# Autodesk Inventor assembly: centre wing
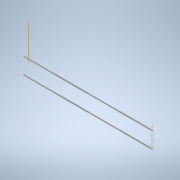
[picture p0: Inventor's stored thumbnail of the model, 180x180]
Saved by Autodesk Inventor 2022 (Build 260153000, 153)
## iProperties
Created: 2021-03-09
Part Number: centre wing
Document SubType Name: Assembly
Designer: Ferdinand Hubbard
Author: Ferdinand Hubbard
## Documents named in this file (4)
- C:\Users\Ferdinand Hubbard\Desktop\solar-plane\cad\centre wing section.iam
- C:\Users\Ferdinand Hubbard\Desktop\solar-plane\cad\18mm tube.ipt
- C:\Users\Ferdinand Hubbard\Desktop\solar-plane\cad\15mm tube.ipt
- C:\Users\Ferdinand Hubbard\Desktop\solar-plane\cad\airfoils\full airfoil\airfoil full 19mm.ipt
## Components (9 placed, 3 different names)
1. 18mm tube:2 — Mate:1, Mate:2, Mate:5, Mate:6
2. 15mm tube:2 — Mate:1, Mate:2
3. 18mm tube:3 — Mate:14, Flush:2
4. 15mm tube:3 — Mate:5, Mate:6
5. 18mm tube:4
6. 15mm tube:4
7. 18mm tube:5 — Mate:13, Flush:1
8. 15mm tube:5
9. airfoil full 19mm:2 — Mate:13, Flush:1, Mate:14, Flush:2
## Relationships (16: Mate 14, Flush 2)
- Mate:1: 18mm tube:2 ↔ 15mm tube:2
- Mate:2: 18mm tube:2 ↔ 15mm tube:2
- [Mate]: 18mm tube:3 ↔ 15mm tube:3
- [Mate]: 18mm tube:3 ↔ 15mm tube:3
- Mate:5: 18mm tube:2 ↔ 15mm tube:3
- Mate:6: 18mm tube:2 ↔ 15mm tube:3
- [Mate]: 18mm tube:4 ↔ 15mm tube:4
- [Mate]: 18mm tube:4 ↔ 15mm tube:4
- [Mate]: 18mm tube:5 ↔ 15mm tube:5
- [Mate]: 18mm tube:5 ↔ 15mm tube:5
- [Mate]: 18mm tube:4 ↔ 15mm tube:5
- [Mate]: 18mm tube:4 ↔ 15mm tube:5
- Mate:13: 18mm tube:5 ↔ airfoil full 19mm:2
- Flush:1: 18mm tube:5 ↔ airfoil full 19mm:2
- Mate:14: 18mm tube:3 ↔ airfoil full 19mm:2
- Flush:2: 18mm tube:3 ↔ airfoil full 19mm:2
## Named parameters: d99_d97 = 0 mm, d100_d98 = 0 mm, d103_d97 = 0 mm, d104_d98 = 0 mm, d105_d99_d97 = 0 mm, d106_d100_d98 = 0 mm, d107_d101 = 0 mm, d108_d102 = 0 mm
